# Autodesk Inventor assembly: castor
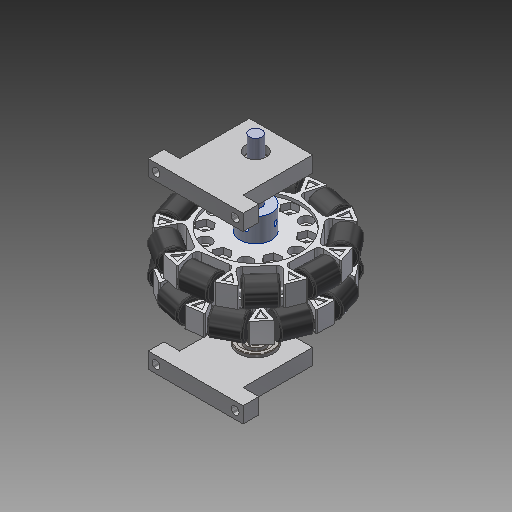
[picture p0: Inventor's stored thumbnail of the model, 512x512]
Saved by Autodesk Inventor 2018 (Build 220112000, 112)
## iProperties
Created: 2017-05-04
Part Number: castor
Document SubType Name: Assembly
Designer: AYUSH SHUKLA
Author: AYUSH SHUKLA
## Documents named in this file (6)
- C:\Study\BTP2\Robomuse Inventor CAD\castor\castor.iam
- C:\Study\BTP2\Robomuse Inventor CAD\castor\castor_shaftfinal.ipt
- C:\Study\BTP2\Robomuse Inventor CAD\castor\castor_bearingfinal.ipt
- C:\Study\BTP2\Robomuse Inventor CAD\castor\radial ball bearing_68_iso_ISO 15 RBB - 108 - 8,SI,NC,8_68.ipt
- C:\Study\BTP2\Robomuse Inventor CAD\castor\final_wheel.iam
- C:\Study\BTP2\Robomuse Inventor CAD\castor\axle.ipt
## Components (8 placed, 5 different names)
1. castor_shaftfinal:1
2. castor_bearingfinal:1
3. radial ball bearing_68_iso_ISO 15 RBB - 108 - 8,SI,NC,8_68:1
4. castor_bearingfinal:2
5. radial ball bearing_68_iso_ISO 15 RBB - 108 - 8,SI,NC,8_68:2
6. final_wheel:1 [sub-assembly]
7. final_wheel:2 [sub-assembly]
8. axle:1
## Relationships (14: Mate 13, Flush 1)
- [Mate]: castor_bearingfinal:1 ↔ radial ball bearing_68_iso_ISO 15 RBB - 108 - 8,SI,NC,8_68:1
- [Mate]: castor_bearingfinal:1 ↔ radial ball bearing_68_iso_ISO 15 RBB - 108 - 8,SI,NC,8_68:1
- [Mate]: castor_shaftfinal:1 ↔ radial ball bearing_68_iso_ISO 15 RBB - 108 - 8,SI,NC,8_68:1
- [Mate]: castor_bearingfinal:2 ↔ radial ball bearing_68_iso_ISO 15 RBB - 108 - 8,SI,NC,8_68:2
- [Mate]: castor_bearingfinal:2 ↔ radial ball bearing_68_iso_ISO 15 RBB - 108 - 8,SI,NC,8_68:2
- [Mate]: castor_shaftfinal:1 ↔ castor_bearingfinal:2
- [Flush] (-9.8 mm): castor_shaftfinal:1 ↔ castor_bearingfinal:2
- [Mate]: final_wheel:1 ↔ final_wheel:2
- [Mate]: final_wheel:1 ↔ final_wheel:2
- [Mate] (10 mm): final_wheel:1 ↔ final_wheel:2
- [Mate]: final_wheel:2 ↔ axle:1
- [Mate]: final_wheel:2 ↔ axle:1
- [Mate]: castor_shaftfinal:1 ↔ axle:1
- [Mate] (33.7 mm): castor_bearingfinal:2 ↔ final_wheel:1
## Named parameters: d52_d49 = 0 mm, d53_d50 = 0 mm
